# Autodesk Inventor assembly: assembly2
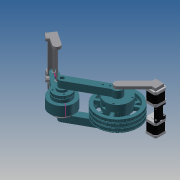
[picture p0: Inventor's stored thumbnail of the model, 180x180]
Saved by Autodesk Inventor 2013 (Build 170138000, 138)
## iProperties
Created: 2017-03-30
Part Number: assembly2
Document SubType Name: Assembly
Designer: employee
Author: employee
## Documents named in this file (23)
- C:\Users\employee\Desktop\SCARA\assembly2.iam
- C:\Users\employee\Desktop\SCARA\stepper.ipt
- C:\Users\employee\Desktop\SCARA\dual stepper mount.ipt
- C:\Users\employee\Desktop\SCARA\M3x8.ipt
- C:\Users\employee\Desktop\SCARA\driven arm.ipt
- C:\Users\employee\Desktop\SCARA\235 drive pulley.ipt
- C:\Users\employee\Desktop\SCARA\layout aide.ipt
- C:\Users\employee\Desktop\SCARA\washer.ipt
- C:\Users\employee\Desktop\SCARA\offset shield.ipt
- C:\Users\employee\Desktop\SCARA\608 bearing.ipt
- C:\Users\employee\Desktop\SCARA\distal idler pulley.ipt
- C:\Users\employee\Desktop\SCARA\z idler pulley.ipt
- C:\Users\employee\Desktop\SCARA\proximal thin arm.ipt
- C:\Users\employee\Desktop\SCARA\distal drive pulley.ipt
- C:\Users\employee\Desktop\SCARA\distal arm.ipt
- C:\Users\employee\Desktop\SCARA\f625.ipt
- C:\Users\employee\Desktop\SCARA\m5 washer.ipt
- C:\Users\employee\Desktop\SCARA\lm6luu.ipt
- C:\Users\employee\Desktop\SCARA\z idler pulley 2.ipt
- C:\Users\employee\Desktop\SCARA\slide frame.ipt
- C:\Users\employee\Desktop\SCARA\rod.ipt
- C:\Users\employee\Desktop\SCARA\stopper.ipt
- C:\Users\employee\Desktop\SCARA\effector.ipt
## Components (52 placed, 22 different names)
1. stepper:1 — Insert:1, Insert:2
2. dual stepper mount:1 — Insert:1, Insert:2, Insert:3, Insert:4, Insert:5, Insert:6, Insert:7, Insert:8, Insert:9, Insert:10
3. stepper:2 — Insert:3, Insert:4, Mate:1, Mate:2
4. M3x8:1 — Insert:8
5. M3x8:2 — Insert:10
6. M3x8:3 — Insert:7
7. M3x8:4 — Insert:9
8. M3x8:5 — Insert:5
9. M3x8:6 — Insert:6
10. layout aide:1 — Mate:1, Mate:2, Insert:11
11. washer:1 — Insert:11, Insert:14
12. offset shield:1 — Insert:15, Mate:3, Insert:16, Insert:17, Insert:18
13. driven arm:1 — Insert:12, Insert:15, Mate:3, Mate:4, Insert:31
14. 608 bearing:2 — Insert:12, Insert:14
15. 608 bearing:3 — Insert:16, Insert:19
16. 235 drive pulley:1 — Insert:17, Insert:18
17. distal idler pulley:1 — Insert:20, Insert:21
18. washer:2 — Insert:19, Insert:22
19. 608 bearing:4 — Insert:20, Insert:22
20. 608 bearing:5 — Insert:21, Insert:23
21. washer:3 — Insert:23, Insert:26
22. z idler pulley:1 — Insert:24, Insert:25
23. washer:5 — Insert:27, Insert:30
24. 608 bearing:6 — Insert:25, Insert:26
25. 608 bearing:7 — Insert:24, Insert:27
26. proximal thin arm:1 — Insert:28, Insert:29, Mate:4, Insert:32
27. 608 bearing:8 — Insert:29
28. 608 bearing:9 — Insert:28, Insert:30
29. washer:6 — Insert:32
30. washer:7 — Insert:31, Insert:34
31. distal drive pulley:1 — Insert:33, Mate:5, Insert:57
32. 608 bearing:10 — Insert:33, Insert:34
33. distal arm:1 — Insert:39, Insert:40, Mate:5, Insert:46, Insert:47, Insert:48, Insert:57
34. f625:1 — Insert:38, Insert:41
35. f625:2 — Insert:36, Insert:42
36. f625:3 — Insert:36
37. f625:4 — Insert:38
38. m5 washer:1 — Insert:40, Insert:42
39. m5 washer:2 — Insert:39, Insert:41
40. lm6luu:1 — Insert:46, Mate:9
41. lm6luu:2 — Insert:47, Mate:8
42. 608 bearing:11 — Insert:48, Insert:49
43. washer:8 — Insert:49, Insert:52
44. z idler pulley 2:1 — Insert:50, Insert:51
45. 608 bearing:12 — Insert:50
46. 608 bearing:13 — Insert:51, Insert:52
47. slide frame:1 — Insert:53, Insert:54, Mate:6, Mate:7, Mate:10, Flush:1, Flush:3
48. rod:1 — Insert:53, Insert:56, Mate:9
49. rod:2 — Insert:54, Insert:55, Mate:8
50. stopper:1 — Insert:55, Mate:7
51. stopper:2 — Insert:56, Mate:6
52. effector:1 — Mate:10, Flush:1, Flush:3
## Relationships (63: Insert 51, Mate 10, Flush 2)
- Insert:1: stepper:1 ↔ dual stepper mount:1
- Insert:2: stepper:1 ↔ dual stepper mount:1
- Insert:3: dual stepper mount:1 ↔ stepper:2
- Insert:4: dual stepper mount:1 ↔ stepper:2
- Insert:5: dual stepper mount:1 ↔ M3x8:5
- Insert:6: dual stepper mount:1 ↔ M3x8:6
- Insert:7: dual stepper mount:1 ↔ M3x8:3
- Insert:8: dual stepper mount:1 ↔ M3x8:1
- Insert:9: dual stepper mount:1 ↔ M3x8:4
- Insert:10: dual stepper mount:1 ↔ M3x8:2
- Mate:1: stepper:2 ↔ layout aide:1
- Mate:2: stepper:2 ↔ layout aide:1
- Insert:11: layout aide:1 ↔ washer:1
- Insert:12: driven arm:1 ↔ 608 bearing:2
- Insert:14: washer:1 ↔ 608 bearing:2
- Insert:15: offset shield:1 ↔ driven arm:1
- Mate:3: offset shield:1 ↔ driven arm:1
- Insert:16: offset shield:1 ↔ 608 bearing:3
- Insert:17: offset shield:1 ↔ 235 drive pulley:1
- Insert:18: offset shield:1 ↔ 235 drive pulley:1
- Insert:19: 608 bearing:3 ↔ washer:2
- Insert:20: distal idler pulley:1 ↔ 608 bearing:4
- Insert:21: distal idler pulley:1 ↔ 608 bearing:5
- Insert:22: washer:2 ↔ 608 bearing:4
- Insert:23: 608 bearing:5 ↔ washer:3
- Insert:24: z idler pulley:1 ↔ 608 bearing:7
- Insert:25: z idler pulley:1 ↔ 608 bearing:6
- Insert:26: washer:3 ↔ 608 bearing:6
- Insert:27: washer:5 ↔ 608 bearing:7
- Insert:28: proximal thin arm:1 ↔ 608 bearing:9
- Insert:29: proximal thin arm:1 ↔ 608 bearing:8
- Insert:30: washer:5 ↔ 608 bearing:9
- Mate:4: driven arm:1 ↔ proximal thin arm:1
- Insert:31: driven arm:1 ↔ washer:7
- Insert:32: proximal thin arm:1 ↔ washer:6
- Insert:33: distal drive pulley:1 ↔ 608 bearing:10
- Insert:34: washer:7 ↔ 608 bearing:10
- Insert:36: f625:2 ↔ f625:3
- Insert:38: f625:1 ↔ f625:4
- Insert:39: distal arm:1 ↔ m5 washer:2
- Insert:40: distal arm:1 ↔ m5 washer:1
- Insert:41: f625:1 ↔ m5 washer:2
- Insert:42: f625:2 ↔ m5 washer:1
- Mate:5: distal drive pulley:1 ↔ distal arm:1
- Insert:46: distal arm:1 ↔ lm6luu:1
- Insert:47: distal arm:1 ↔ lm6luu:2
- Insert:48: distal arm:1 ↔ 608 bearing:11
- Insert:49: 608 bearing:11 ↔ washer:8
- Insert:50: z idler pulley 2:1 ↔ 608 bearing:12
- Insert:51: z idler pulley 2:1 ↔ 608 bearing:13
- Insert:52: washer:8 ↔ 608 bearing:13
- Insert:53: slide frame:1 ↔ rod:1
- Insert:54: slide frame:1 ↔ rod:2
- Insert:55: rod:2 ↔ stopper:1
- Insert:56: rod:1 ↔ stopper:2
- Mate:6: slide frame:1 ↔ stopper:2
- Mate:7: slide frame:1 ↔ stopper:1
- Mate:8: lm6luu:2 ↔ rod:2
- Mate:9: lm6luu:1 ↔ rod:1
- Mate:10: slide frame:1 ↔ effector:1
- Flush:1: slide frame:1 ↔ effector:1
- Insert:57: distal drive pulley:1 ↔ distal arm:1
- Flush:3 (-0.9 mm): slide frame:1 ↔ effector:1
